# Autodesk Inventor assembly: OdometryAssembly
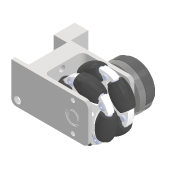
[picture p0: Inventor's stored thumbnail of the model, 180x180]
Saved by Autodesk Inventor 2020 (Build 240168000, 168)
## iProperties
Created: 2019-07-05
Part Number: OdometryAssembly
Document SubType Name: Assembly
Designer: ishaa
Author: ishaa
## Documents named in this file (9)
- C:\FTC\FTC8863CAD\2019 Robot\Odoemetry module\OdometryAssembly.iam
- C:\FTC\FTC8863CAD\2019 Robot\Odoemetry module\Odometry_Holder.ipt
- C:\FTC\FTC8863CAD\2019 Robot\Odoemetry module\E8T-X-236-S-D-M-X.ipt
- C:\FTC\FTC8863CAD\Actobotics\535 parts\535042.ipt
- C:\FTC\FTC8863CAD\2019 Robot\Odoemetry module\14166.iam
- C:\FTC\FTC8863CAD\2019 Robot\Odoemetry module\90576A161_MEDIUM-STRENGTH STEEL NYLON-INSERT LOCKNUT.ipt
- C:\FTC\FTC8863CAD\2019 Robot\Odoemetry module\spacerBigOdometry.ipt
- C:\FTC\FTC8863CAD\2019 Robot\Odoemetry module\spacerSmallOdometry.ipt
- C:\FTC\FTC8863CAD\Actobotics\634 parts\634064.ipt
## Components (10 placed, 8 different names)
1. Odometry_Holder:1 — Insert:1, Mate:1, Insert:2, Insert:3, Insert:4, Insert:5, Flush:1
2. E8T-X-236-S-D-M-X:1 — Insert:1, Mate:1
3. 535042:1 — Insert:2, Insert:6
4. 535042:2 — Insert:3, Mate:2, Insert:7, Mate:4
5. 14166:1 [sub-assembly] — Mate:2, Mate:3
6. 90576A161_MEDIUM-STRENGTH STEEL NYLON-INSERT LOCKNUT:1 — Insert:4
7. 90576A161_MEDIUM-STRENGTH STEEL NYLON-INSERT LOCKNUT:2 — Insert:5
8. spacerBigOdometry:1 — Insert:6, Mate:3
9. spacerSmallOdometry:1 — Insert:7
10. 634064:1 — Mate:4, Flush:1
## Relationships (12: Insert 7, Mate 4, Flush 1)
- Insert:1: Odometry_Holder:1 ↔ E8T-X-236-S-D-M-X:1
- Mate:1: Odometry_Holder:1 ↔ E8T-X-236-S-D-M-X:1
- Insert:2: Odometry_Holder:1 ↔ 535042:1
- Insert:3: Odometry_Holder:1 ↔ 535042:2
- Mate:2: 535042:2 ↔ 14166:1
- Insert:4: Odometry_Holder:1 ↔ 90576A161_MEDIUM-STRENGTH STEEL NYLON-INSERT LOCKNUT:1
- Insert:5: Odometry_Holder:1 ↔ 90576A161_MEDIUM-STRENGTH STEEL NYLON-INSERT LOCKNUT:2
- Insert:6: 535042:1 ↔ spacerBigOdometry:1
- Mate:3: 14166:1 ↔ spacerBigOdometry:1
- Insert:7: 535042:2 ↔ spacerSmallOdometry:1
- Mate:4: 535042:2 ↔ 634064:1
- Flush:1: Odometry_Holder:1 ↔ 634064:1
